# Autodesk Inventor assembly: Złożenie ramienia robota
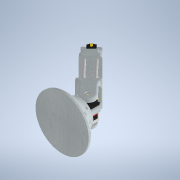
[picture p0: Inventor's stored thumbnail of the model, 180x180]
Saved by Autodesk Inventor 2021 (Build 250183000, 183)
## iProperties
Created: 2021-11-03
Part Number: Złożenie ramienia robota
Document SubType Name: Assembly
Designer: Łukasz
Author: Łukasz
## Documents named in this file (14)
- E:\GITHUB_Czołg\Szybki-Czolg-antyRadziecki\Ramie robota\Ramie robota\Złożenie ramienia robota.iam
- E:\GITHUB_Czołg\Szybki-Czolg-antyRadziecki\Ramie robota\Ramie robota\Podstawa 01-1.ipt
- E:\GITHUB_Czołg\Szybki-Czolg-antyRadziecki\Ramie robota\Ramie robota\Podstawa 01-2.ipt
- E:\GITHUB_Czołg\Szybki-Czolg-antyRadziecki\Ramie robota\Ramie robota\serwo 30x70.ipt
- E:\GITHUB_Czołg\Szybki-Czolg-antyRadziecki\Ramie robota\Ramie robota\mocowanie lozyska 10-1.ipt
- C:\Users\Łukasz\Documents\Inventor\Content Center Files\R2021\en-US\BS 292 (I)\BS 292 Part 1 - 608 - 8 x 22 x 7.ipt
- E:\GITHUB_Czołg\Szybki-Czolg-antyRadziecki\Ramie robota\Ramie robota\orczyk serwa okrągły 02-1.ipt
- E:\GITHUB_Czołg\Szybki-Czolg-antyRadziecki\Ramie robota\Ramie robota\ramie 03-1.ipt
- C:\Users\Łukasz\Documents\Inventor\Content Center Files\R2021\en-US\AS 1427(02)\AS 1427 - M8 x 16(2).ipt
- E:\GITHUB_Czołg\Szybki-Czolg-antyRadziecki\Ramie robota\Ramie robota\pręt 04-1.ipt
- E:\GITHUB_Czołg\Szybki-Czolg-antyRadziecki\Ramie robota\Ramie robota\podstawa 01-3.ipt
- E:\GITHUB_Czołg\Szybki-Czolg-antyRadziecki\Ramie robota\Ramie robota\servo 20x40.ipt
- E:\GITHUB_Czołg\Szybki-Czolg-antyRadziecki\Ramie robota\Ramie robota\ramie 03-2.ipt
- E:\GITHUB_Czołg\Szybki-Czolg-antyRadziecki\Ramie robota\Ramie robota\ramie 03-3.ipt
## Components (16 placed, 13 different names)
1. Podstawa 01-1:1 — Mate:1, Mate:2, Mate:3
2. Podstawa 01-2:1 — Mate:4, Mate:5, Mate:6
3. serwo 30x70:1 — Mate:1, Mate:2, Mate:3, Mate:4, Mate:5, Mate:6, Mate:7, Flush:2, Rotational:2, Mate:8, Mate:9, Mate:10, Mate:11
4. mocowanie lozyska 10-1:1 — Mate:7, Flush:2, Rotational:1, Mate:8
5. BS 292: Part 1 (I) (Metric) 608 - 8 x 22 x 7:1 — Rotational:1
6. orczyk serwa okrągły 02-1:1 — Rotational:2, Rotational:3
7. ramie 03-1:1 — Rotational:3, Rotational:4, Rigid:1, Rigid:2, Rigid:3, Rigid:4
8. AS 1427 - Metric M8 x 16:1 — Rotational:4
9. pręt 04-1:1 — Rigid:1, Rotational:6
10. pręt 04-1:2 — Rigid:2, Rotational:5
11. pręt 04-1:3 — Rigid:3
12. pręt 04-1:4 — Rigid:4
13. podstawa 01-3:1 — Mate:9, Mate:10, Mate:11
14. servo 20x40:1 — Mate:12, Mate:13, Mate:14, Mate:15
15. ramie 03-2:1 — Mate:12, Mate:13, Mate:14, Rotational:5, Rotational:6, Flush:3, Flush:4
16. ramie 03-3:1 — Mate:15, Flush:3, Flush:4
## Relationships (28: Mate 15, RevoluteJoint 6, WeldJoint 4, Flush 3)
- Mate:1: Podstawa 01-1:1 ↔ serwo 30x70:1
- Mate:2: Podstawa 01-1:1 ↔ serwo 30x70:1
- Mate:3: Podstawa 01-1:1 ↔ serwo 30x70:1
- Mate:4: Podstawa 01-2:1 ↔ serwo 30x70:1
- Mate:5: Podstawa 01-2:1 ↔ serwo 30x70:1
- Mate:6: Podstawa 01-2:1 ↔ serwo 30x70:1
- Mate:7: serwo 30x70:1 ↔ mocowanie lozyska 10-1:1
- Flush:2: serwo 30x70:1 ↔ mocowanie lozyska 10-1:1
- Rotational:1 [RevoluteJoint]: mocowanie lozyska 10-1:1 ↔ BS 292: Part 1 (I) (Metric) 608 - 8 x 22 x 7:1
- Rotational:2 [RevoluteJoint]: serwo 30x70:1 ↔ orczyk serwa okrągły 02-1:1
- Mate:8: serwo 30x70:1 ↔ mocowanie lozyska 10-1:1
- Rotational:3 [RevoluteJoint]: orczyk serwa okrągły 02-1:1 ↔ ramie 03-1:1
- Rotational:4 [RevoluteJoint]: ramie 03-1:1 ↔ AS 1427 - Metric M8 x 16:1
- Rigid:1 [WeldJoint] (5 mm): ramie 03-1:1 ↔ pręt 04-1:1
- Rigid:2 [WeldJoint] (5 mm): ramie 03-1:1 ↔ pręt 04-1:2
- Rigid:3 [WeldJoint] (5 mm): ramie 03-1:1 ↔ pręt 04-1:3
- Rigid:4 [WeldJoint] (5 mm): ramie 03-1:1 ↔ pręt 04-1:4
- Mate:9: serwo 30x70:1 ↔ podstawa 01-3:1
- Mate:10: serwo 30x70:1 ↔ podstawa 01-3:1
- Mate:11: serwo 30x70:1 ↔ podstawa 01-3:1
- Mate:12: servo 20x40:1 ↔ ramie 03-2:1
- Mate:13: servo 20x40:1 ↔ ramie 03-2:1
- Mate:14: servo 20x40:1 ↔ ramie 03-2:1
- Rotational:5 [RevoluteJoint]: pręt 04-1:2 ↔ ramie 03-2:1
- Rotational:6 [RevoluteJoint]: pręt 04-1:1 ↔ ramie 03-2:1
- Mate:15: servo 20x40:1 ↔ ramie 03-3:1
- Flush:3: ramie 03-2:1 ↔ ramie 03-3:1
- Flush:4: ramie 03-2:1 ↔ ramie 03-3:1
